# Autodesk Inventor assembly: Main Assembly
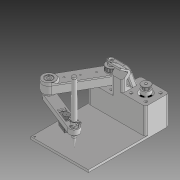
[picture p0: Inventor's stored thumbnail of the model, 180x180]
Saved by Autodesk Inventor 2020 (Build 240168000, 168)
## iProperties
Created: 2020-07-24
Part Number: Main Assembly
Document SubType Name: Assembly
Designer: DDeGo
Author: DDeGo
## Documents named in this file (12)
- C:\Users\DDeGo\Documents\Drew\Projects\Tic Tac Toe Bot\cad\Main Assembly.iam
- C:\Users\DDeGo\Documents\Drew\Projects\Tic Tac Toe Bot\cad\Base.ipt
- C:\Users\DDeGo\Documents\Drew\Projects\Tic Tac Toe Bot\cad\GT2 20T Drive Pulley.ipt
- C:\Users\DDeGo\Documents\Drew\Projects\Tic Tac Toe Bot\cad\GT2 Idler Pulley.ipt
- C:\Users\DDeGo\Documents\Drew\Projects\Tic Tac Toe Bot\cad\Nema 17.ipt
- C:\Users\DDeGo\Documents\Drew\Projects\Tic Tac Toe Bot\cad\Scara1.ipt
- C:\Users\DDeGo\Documents\Drew\Projects\Tic Tac Toe Bot\cad\625 Bearing.ipt
- C:\Users\DDeGo\Documents\Drew\Projects\Tic Tac Toe Bot\cad\Scara1_top.ipt
- C:\Users\DDeGo\Documents\Drew\Projects\Tic Tac Toe Bot\cad\Scara2.ipt
- C:\Users\DDeGo\Documents\Drew\Projects\Tic Tac Toe Bot\cad\MG90servo_body.ipt
- C:\Users\DDeGo\Documents\Drew\Projects\Tic Tac Toe Bot\cad\pen.ipt
- C:\Users\DDeGo\Documents\Drew\Projects\Tic Tac Toe Bot\cad\Pen Sleeve.ipt
## Components (16 placed, 11 different names)
1. Base:1 — Mate:2, Mate:3, Mate:4, Mate:5, Mate:6, Mate:10, Mate:33
2. GT2 Idler Pulley:1 — Mate:8, Rotation:2
3. Nema 17:1 — Mate:4, Mate:6, Mate:10, Mate:14
4. Scara1:1 — Mate:34, Mate:35, Mate:36, Mate:37, Mate:42, Mate:43, Mate:44, Mate:45, Mate:47
5. Nema 17:2 — Mate:2, Mate:3, Mate:5, Mate:8, Mate:31, Mate:45
6. GT2 Idler Pulley:2 — Rotation:2, Mate:46, Mate:47
7. GT2 20T Drive Pulley:1 — Mate:14, Flush:1, Rotation:1
8. 625 Bearing:1 — Mate:31, Mate:40, Mate:41
9. 625 Bearing:2 — Mate:34, Mate:35
10. 625 Bearing:3 — Mate:36, Mate:37, Mate:38, Mate:39
11. 625 Bearing:4 — Mate:20, Mate:22, Mate:46
12. Scara1_top:1 — Mate:20, Mate:22, Flush:1, Rotation:1, Mate:40, Mate:41, Mate:42, Mate:43, Mate:44
13. Scara2:1 — Mate:26, Mate:27, Angle:1, Mate:28, Mate:38, Mate:39
14. MG90servo_body:1 — Mate:26, Mate:27, Angle:1
15. pen:1 — Mate:28, Mate:29, Mate:30, Mate:33
16. Pen Sleeve:1 — Mate:29, Mate:30
## Relationships (35: Mate 31, RelateRotation 2, Angle 1, Flush 1)
- Mate:2: Base:1 ↔ Nema 17:2
- Mate:3: Base:1 ↔ Nema 17:2
- Mate:4: Base:1 ↔ Nema 17:1
- Mate:5: Base:1 ↔ Nema 17:2
- Mate:6: Base:1 ↔ Nema 17:1
- Mate:8: GT2 Idler Pulley:1 ↔ Nema 17:2
- Mate:10: Base:1 ↔ Nema 17:1
- Mate:14: Nema 17:1 ↔ GT2 20T Drive Pulley:1
- Mate:20: 625 Bearing:4 ↔ Scara1_top:1
- Mate:22: 625 Bearing:4 ↔ Scara1_top:1
- Mate:26: Scara2:1 ↔ MG90servo_body:1
- Mate:27: Scara2:1 ↔ MG90servo_body:1
- Angle:1 (0 deg): Scara2:1 ↔ MG90servo_body:1
- Mate:28: Scara2:1 ↔ pen:1
- Mate:29: pen:1 ↔ Pen Sleeve:1
- Mate:30: pen:1 ↔ Pen Sleeve:1
- Flush:1: GT2 20T Drive Pulley:1 ↔ Scara1_top:1
- Rotation:1 [RelateRotation] (1.8 ul): GT2 20T Drive Pulley:1 ↔ Scara1_top:1
- Rotation:2 [RelateRotation] (1 ul): GT2 Idler Pulley:1 ↔ GT2 Idler Pulley:2
- Mate:31: Nema 17:2 ↔ 625 Bearing:1
- Mate:33: Base:1 ↔ pen:1
- Mate:34: Scara1:1 ↔ 625 Bearing:2
- Mate:35: Scara1:1 ↔ 625 Bearing:2
- Mate:36: Scara1:1 ↔ 625 Bearing:3
- Mate:37: Scara1:1 ↔ 625 Bearing:3
- Mate:38: 625 Bearing:3 ↔ Scara2:1
- Mate:39 (1 mm): 625 Bearing:3 ↔ Scara2:1
- Mate:40: 625 Bearing:1 ↔ Scara1_top:1
- Mate:41: 625 Bearing:1 ↔ Scara1_top:1
- Mate:42: Scara1:1 ↔ Scara1_top:1
- Mate:43: Scara1:1 ↔ Scara1_top:1
- Mate:44: Scara1:1 ↔ Scara1_top:1
- Mate:45 (2 mm): Scara1:1 ↔ Nema 17:2
- Mate:46: GT2 Idler Pulley:2 ↔ 625 Bearing:4
- Mate:47 (1 mm): Scara1:1 ↔ GT2 Idler Pulley:2
